# Autodesk Inventor assembly: Crank_Slider_Fixer
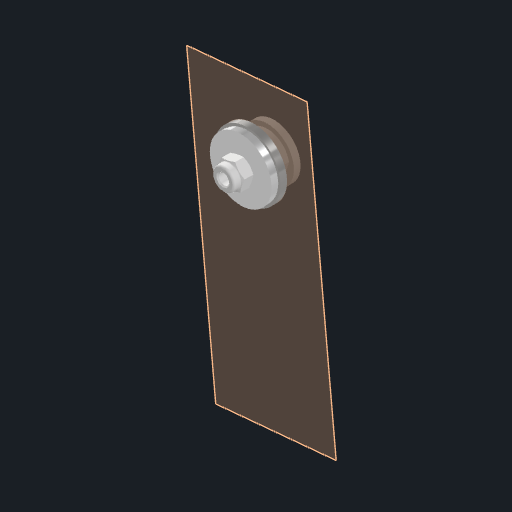
[picture p0: Inventor's stored thumbnail of the model, 512x512]
Saved by Autodesk Inventor 2024.3 (Build 283343000, 343)
## iProperties
Created: 2024-01-28
Part Number: Crank_Slider_Fixer
Document SubType Name: Assembly
Designer: 김대겸
Author: 김대겸
## Documents named in this file (5)
- C:\Users\ASUS\Desktop\test\v2_Frame\Crank_Slider_Fixer.iam
- C:\Users\ASUS\Desktop\test\v1_Frame\MISUMI\LED-0606.ipt
- C:\Users\ASUS\Desktop\test\v2_Frame\MISUMI\W1SSS15-10-1.5.ipt
- C:\Users\ASUS\Desktop\test\v2_Frame\Handmade tiered cover_9mm_Wide_ALU.ipt
- C:\Users\ASUS\Desktop\test\v2_Frame\MISUMI\K1148.ipt
## Components (4 placed, 4 different names)
1. LED-0606:1 — 메이트:6, 메이트:7
2. W1SSS15-10-1.5:1 — 메이트:6, 메이트:7, 삽입:2
3. Handmade tiered cover_9mm_Wide_ALU:2 — 삽입:2, 삽입:3
4. K1148:1 — 삽입:3
## Relationships (4: Mate 2, Insert 2)
- 메이트:6 [Mate] (3 mm): LED-0606:1 ↔ W1SSS15-10-1.5:1
- 메이트:7 [Mate]: LED-0606:1 ↔ W1SSS15-10-1.5:1
- 삽입:2 [Insert]: W1SSS15-10-1.5:1 ↔ Handmade tiered cover_9mm_Wide_ALU:2
- 삽입:3 [Insert]: Handmade tiered cover_9mm_Wide_ALU:2 ↔ K1148:1
